# Autodesk Inventor assembly: WCP DS Gearbox
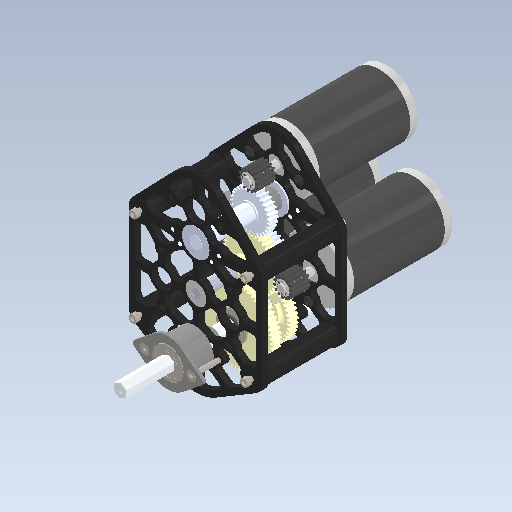
[picture p0: Inventor's stored thumbnail of the model, 512x512]
Saved by Autodesk Inventor 2020 (Build 240168000, 168)
## iProperties
Created: 2013-12-10
Part Number: WCP DS Gearbox
Description: STEP AP214
Document SubType Name: Assembly
Designer: aidan
Sending System: SolidWorks 2013
Preprocessor: SwSTEP 2.0
Title: 217-3433-STEP.STEP
Revision Number: ANY
## Documents named in this file (44)
- C:\Users\aidan\Desktop\T3 Robotics\CAD\WCP DS Gearbox.iam
- C:\Users\aidan\Desktop\T3 Robotics\CAD\WCP DS Gearbox\217-2428-027 Rev1_97414A630.ipt
- C:\Users\aidan\Desktop\T3 Robotics\CAD\WCP DS Gearbox\217-3423-005 Rev1.ipt
- C:\Users\aidan\Desktop\T3 Robotics\CAD\WCP DS Gearbox\217-3195-200 Rev1.iam
- C:\Users\aidan\Desktop\T3 Robotics\CAD\WCP DS Gearbox\217-3489.ipt
- C:\Users\aidan\Desktop\T3 Robotics\CAD\WCP DS Gearbox\217-3423-006 Rev1.ipt
- C:\Users\aidan\Desktop\T3 Robotics\CAD\WCP DS Gearbox\217-3423-008 Rev1.ipt
- C:\Users\aidan\Desktop\T3 Robotics\CAD\WCP DS Gearbox\217-3423-009 Rev1.ipt
- C:\Users\aidan\Desktop\T3 Robotics\CAD\WCP DS Gearbox\217-2778-001 Rev2_NCQ8A075-050M.iam
- C:\Users\aidan\Desktop\T3 Robotics\CAD\WCP DS Gearbox\217-2731.ipt
- C:\Users\aidan\Desktop\T3 Robotics\CAD\WCP DS Gearbox\217-2733.ipt
- C:\Users\aidan\Desktop\T3 Robotics\CAD\WCP DS Gearbox\217-2734.ipt
- C:\Users\aidan\Desktop\T3 Robotics\CAD\WCP DS Gearbox\217-2743.ipt
- C:\Users\aidan\Desktop\T3 Robotics\CAD\WCP DS Gearbox\217-2614-002_98430A132.ipt
- C:\Users\aidan\Desktop\T3 Robotics\CAD\WCP DS Gearbox\217-3421-007 Rev1.ipt
- C:\Users\aidan\Desktop\T3 Robotics\CAD\WCP DS Gearbox\217-3421-009 Rev1.ipt
- C:\Users\aidan\Desktop\T3 Robotics\CAD\WCP DS Gearbox\217-3421-010 Rev1.ipt
- C:\Users\aidan\Desktop\T3 Robotics\CAD\WCP DS Gearbox\217-3421-011 Rev2_97633A200.ipt
- C:\Users\aidan\Desktop\T3 Robotics\CAD\WCP DS Gearbox\217-3422-007 Rev1.ipt
- C:\Users\aidan\Desktop\T3 Robotics\CAD\WCP DS Gearbox\217-3423-014 Rev1.ipt
- C:\Users\aidan\Desktop\T3 Robotics\CAD\WCP DS Gearbox\217-3423-016 Rev1.ipt
- C:\Users\aidan\Desktop\T3 Robotics\CAD\WCP DS Gearbox\217-3424-003 Rev1.ipt
- C:\Users\aidan\Desktop\T3 Robotics\CAD\WCP DS Gearbox\217-2761-001 rev1.ipt
- C:\Users\aidan\Desktop\T3 Robotics\CAD\WCP DS Gearbox\217-3210-001 Rev1_30t.ipt
- C:\Users\aidan\Desktop\T3 Robotics\CAD\WCP DS Gearbox\217-3215-001 Rev1_42t.ipt
- C:\Users\aidan\Desktop\T3 Robotics\CAD\WCP DS Gearbox\217-3414-001 Rev1_14t Steel Pinion.ipt
- C:\Users\aidan\Desktop\T3 Robotics\CAD\WCP DS Gearbox\217-3418-001 Rev2_44t.ipt
- C:\Users\aidan\Desktop\T3 Robotics\CAD\WCP DS Gearbox\217-3420-001 Rev2_60t.ipt
- C:\Users\aidan\Desktop\T3 Robotics\CAD\WCP DS Gearbox\217-3100-001_14t.ipt
- C:\Users\aidan\Desktop\T3 Robotics\CAD\WCP DS Gearbox\217-2705-001_30t.ipt
- C:\Users\aidan\Desktop\T3 Robotics\CAD\WCP DS Gearbox\217-2000.ipt
- C:\Users\aidan\Desktop\T3 Robotics\CAD\WCP DS Gearbox\217-3433-001 Rev1_Default_As Machined_.ipt
- C:\Users\aidan\Desktop\T3 Robotics\CAD\WCP DS Gearbox\217-3423-003 Rev1.ipt
- C:\Users\aidan\Desktop\T3 Robotics\CAD\WCP DS Gearbox\217-3424-005 Rev1.ipt
- C:\Users\aidan\Desktop\T3 Robotics\CAD\WCP DS Gearbox\217-3433-003 Rev1.ipt
- C:\Users\aidan\Desktop\T3 Robotics\CAD\WCP DS Gearbox\217-3256-001 Rev1.ipt
- C:\Users\aidan\Desktop\T3 Robotics\CAD\WCP DS Gearbox\217-3261-001 Rev1.ipt
- C:\Users\aidan\Desktop\T3 Robotics\CAD\WCP DS Gearbox\217-3423-004 Rev1.ipt
- C:\Users\aidan\Desktop\T3 Robotics\CAD\WCP DS Gearbox\217-3424-002 Rev1.ipt
- C:\Users\aidan\Desktop\T3 Robotics\CAD\WCP DS Gearbox\217-3422-004 Rev2.ipt
- C:\Users\aidan\Desktop\T3 Robotics\CAD\WCP DS Gearbox\217-3257-001 Rev1.ipt
- C:\Users\aidan\Desktop\T3 Robotics\CAD\WCP DS Gearbox\217-3263-001 Rev1.ipt
- C:\Users\aidan\Desktop\T3 Robotics\CAD\WCP DS Gearbox\217-3259-001 Rev1.ipt
- C:\Users\aidan\Desktop\T3 Robotics\CAD\WCP DS Gearbox\217-2758-001 Rev1.ipt
## Components (78 placed, 78 different names)
1. 217-2428-027 Rev1_97414A630_1
2. 217-3423-005 Rev1_2
3. 217-3195-200 Rev1_3 [sub-assembly]
4. 217-3489_4
5. 217-3423-006 Rev1_5
6. 217-3423-006 Rev1_6
7. 217-3423-008 Rev1_7
8. 217-3423-009 Rev1_8
9. 217-2778-001 Rev2_NCQ8A075-050M_9 [sub-assembly]
10. 217-2731_10
11. 217-2733_11
12. 217-2733_12
13. 217-2734_13 — Mate:1, Mate:2, Mate:5, Mate:6, Mate:7
14. 217-2734_14
15. 217-2743_15
16. 217-2731_16
17. 217-2731_17
18. 217-2614-002_98430A132_18
19. 217-2614-002_98430A132_19
20. 217-2614-002_98430A132_20
21. 217-2614-002_98430A132_21
22. 217-2614-002_98430A132_22
23. 217-2614-002_98430A132_23
24. 217-3421-007 Rev1_24
25. 217-3421-007 Rev1_25
26. 217-3421-009 Rev1_26
27. 217-3421-009 Rev1_27
28. 217-3421-009 Rev1_28
29. 217-3421-009 Rev1_29
30. 217-3421-009 Rev1_30
31. 217-3421-009 Rev1_31
32. 217-3421-010 Rev1_32
33. 217-3421-010 Rev1_33
34. 217-3421-010 Rev1_34
35. 217-3421-010 Rev1_35
36. 217-3421-011 Rev2_97633A200_36 — Mate:8
37. 217-3422-007 Rev1_37
38. 217-3422-007 Rev1_38
39. 217-3423-014 Rev1_39
40. 217-3423-016 Rev1_40
41. 217-3423-016 Rev1_41
42. 217-3423-016 Rev1_42
43. 217-3424-003 Rev1_43
44. 217-3424-003 Rev1_44
45. 217-3424-003 Rev1_45
46. 217-3424-003 Rev1_46
47. 217-2761-001 rev1_47
48. 217-2761-001 rev1_48
49. 217-2761-001 rev1_49
50. 217-3210-001 Rev1_30t_50
51. 217-3215-001 Rev1_42t_51
52. 217-3414-001 Rev1_14t Steel Pinion_52
53. 217-3414-001 Rev1_14t Steel Pinion_53
54. 217-3414-001 Rev1_14t Steel Pinion_54
55. 217-3418-001 Rev2_44t_55
56. 217-3420-001 Rev2_60t_56
57. 217-3100-001_14t_57
58. 217-2705-001_30t_58
59. 217-2000_59
60. 217-2000_60
61. 217-2000_61
62. 217-3433-001 Rev1_Default<As Machined>_62
63. 217-3433-001 Rev1_Default<As Machined>_63
64. 217-3423-003 Rev1_64 — Mate:1, Mate:2, Mate:3, Mate:4, Mate:8
65. 217-3424-005 Rev1_65
66. 217-3433-003 Rev1_66
67. 217-3256-001 Rev1_67
68. 217-3261-001 Rev1_68
69. 217-3423-004 Rev1_69
70. 217-3424-002 Rev1_70
71. 217-3424-002 Rev1_71
72. 217-3424-002 Rev1_72
73. 217-3424-002 Rev1_73
74. 217-3422-004 Rev2_74 — Mate:6, Mate:7
75. 217-3257-001 Rev1_75
76. 217-3263-001 Rev1_76 — Mate:3, Mate:4, Mate:5
77. 217-3259-001 Rev1_77
78. 217-2758-001 Rev1_78
## Relationships (8: Mate 8)
- Mate:1: 217-2734_13 ↔ 217-3423-003 Rev1_64
- Mate:2: 217-2734_13 ↔ 217-3423-003 Rev1_64
- Mate:3: 217-3423-003 Rev1_64 ↔ 217-3263-001 Rev1_76
- Mate:4: 217-3423-003 Rev1_64 ↔ 217-3263-001 Rev1_76
- Mate:5: 217-2734_13 ↔ 217-3263-001 Rev1_76
- Mate:6: 217-2734_13 ↔ 217-3422-004 Rev2_74
- Mate:7: 217-2734_13 ↔ 217-3422-004 Rev2_74
- Mate:8: 217-3421-011 Rev2_97633A200_36 ↔ 217-3423-003 Rev1_64
